# Autodesk Inventor assembly: esp_case_assy
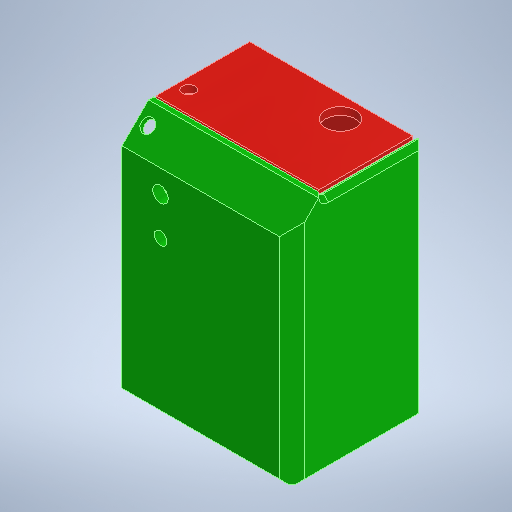
[picture p0: Inventor's stored thumbnail of the model, 512x512]
Saved by Autodesk Inventor 2025 (Build 290162000, 162)
## iProperties
Created: 2025-03-25
Part Number: esp_case_assy
Document SubType Name: Assembly
Designer: VianaCC
Author: VianaCC
## Documents named in this file (3)
- C:\Users\vianacc\Documents\esp_case_assy.iam
- C:\Users\vianacc\Documents\ESP_case2.ipt
- C:\Users\vianacc\Documents\ESP_case1.ipt
## Components (2 placed, 2 different names)
1. ESP_case2:1 — Mate:2, Mate:3, Mate:4
2. ESP_case1:1 — Mate:1, Mate:2, Mate:3, Mate:4
## Relationships (4: Mate 4)
- Mate:1: ESP_case1:1
- Mate:2 (0.1 mm): ESP_case2:1 ↔ ESP_case1:1
- Mate:3 (0.1 mm): ESP_case2:1 ↔ ESP_case1:1
- Mate:4: ESP_case2:1 ↔ ESP_case1:1
